# Autodesk Inventor assembly: frame assembly 4
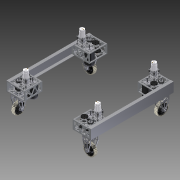
[picture p0: Inventor's stored thumbnail of the model, 180x180]
Saved by Autodesk Inventor 2012 (Build 160160000, 160)
## iProperties
Created: 2013-07-06
Part Number: frame assembly 4
Document SubType Name: Assembly
Designer: Bryce
Author: Bryce
## Documents named in this file (3)
- C:\Users\Bryce\Dropbox\Inventor Design Project Files\Independent Swerves\Inventor 2012\frame assembly 4.iam
- C:\Users\Bryce\Dropbox\Inventor Design Project Files\Independent Swerves\Inventor 2012\FULL SWERVE DRIVE ASSEMBLY!  2!.iam
- C:\Users\Bryce\Dropbox\Inventor Design Project Files\Independent Swerves\Inventor 2012\big U channel 3.25in.ipt
## Components (6 placed, 2 different names)
1. FULL SWERVE DRIVE ASSEMBLY!  2!:1 [sub-assembly] — Mate:1, Flush:1, Mate:2, Flush:6
2. FULL SWERVE DRIVE ASSEMBLY!  2!:2 [sub-assembly] — Mate:7, Mate:8, Flush:4
3. FULL SWERVE DRIVE ASSEMBLY!  2!:3 [sub-assembly] — Mate:3, Mate:4, Flush:2, Flush:5
4. FULL SWERVE DRIVE ASSEMBLY!  2!:4 [sub-assembly] — Flush:3, Mate:5, Mate:6, Flush:5, Flush:6
5. big U channel 3.25in:1 — Mate:1, Flush:1, Mate:2, Mate:3, Mate:4, Flush:2
6. big U channel 3.25in:2 — Flush:3, Mate:5, Mate:6, Mate:7, Mate:8, Flush:4
## Relationships (14: Mate 8, Flush 6)
- Mate:1: FULL SWERVE DRIVE ASSEMBLY!  2!:1 ↔ big U channel 3.25in:1
- Flush:1: FULL SWERVE DRIVE ASSEMBLY!  2!:1 ↔ big U channel 3.25in:1
- Mate:2: FULL SWERVE DRIVE ASSEMBLY!  2!:1 ↔ big U channel 3.25in:1
- Mate:3: FULL SWERVE DRIVE ASSEMBLY!  2!:3 ↔ big U channel 3.25in:1
- Mate:4: FULL SWERVE DRIVE ASSEMBLY!  2!:3 ↔ big U channel 3.25in:1
- Flush:2: FULL SWERVE DRIVE ASSEMBLY!  2!:3 ↔ big U channel 3.25in:1
- Flush:3: FULL SWERVE DRIVE ASSEMBLY!  2!:4 ↔ big U channel 3.25in:2
- Mate:5: FULL SWERVE DRIVE ASSEMBLY!  2!:4 ↔ big U channel 3.25in:2
- Mate:6: FULL SWERVE DRIVE ASSEMBLY!  2!:4 ↔ big U channel 3.25in:2
- Mate:7: FULL SWERVE DRIVE ASSEMBLY!  2!:2 ↔ big U channel 3.25in:2
- Mate:8: FULL SWERVE DRIVE ASSEMBLY!  2!:2 ↔ big U channel 3.25in:2
- Flush:4: FULL SWERVE DRIVE ASSEMBLY!  2!:2 ↔ big U channel 3.25in:2
- Flush:5: FULL SWERVE DRIVE ASSEMBLY!  2!:3 ↔ FULL SWERVE DRIVE ASSEMBLY!  2!:4
- Flush:6: FULL SWERVE DRIVE ASSEMBLY!  2!:1 ↔ FULL SWERVE DRIVE ASSEMBLY!  2!:4
